# Autodesk Inventor assembly: Synchronous Belts Transmission
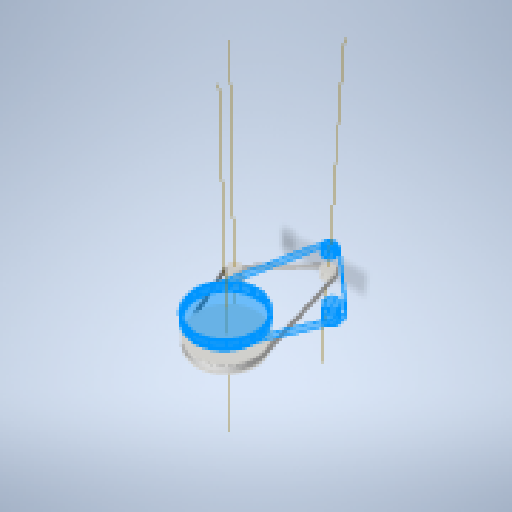
[picture p0: Inventor's stored thumbnail of the model, 512x512]
Saved by Autodesk Inventor 2024 (Build 280153000, 153)
## iProperties
ClientObjectVersion: 1
Created: 2024-01-05
Part Number: Synchronous Belts Transmission
Document SubType Name: Assembly
Designer: MaartenGeorgesBuelen
Author: MaartenGeorgesBuelen
## Documents named in this file (5)
- C:\Users\MaartenGeorgesBuelen\Documents\Inventor\robot arm\base\Design Accelerator\Synchronous Belts Transmission3.iam
- C:\Users\MaartenGeorgesBuelen\Documents\Inventor\robot arm\base\Design Accelerator\Synchronous Belt3.ipt
- C:\Users\MaartenGeorgesBuelen\Documents\Inventor\robot arm\base\Design Accelerator\Synchronous Pulley13.ipt
- C:\Users\MaartenGeorgesBuelen\Documents\Inventor\robot arm\base\Design Accelerator\Synchronous Pulley23.ipt
- C:\Users\MaartenGeorgesBuelen\Documents\Inventor\robot arm\base\Design Accelerator\Synchronous Pulley32.ipt
## Components (4 placed, 4 different names)
1. Synchronous Belt:1 — Flush:1, Mate:1, Mate:2, Flush:2, Mate:3, Mate:4, Flush:3, Mate:5, Mate:6
2. Synchronous Pulley1:1 — Flush:1, Mate:1, Mate:2, Rotation:1, Rotation:2
3. Synchronous Pulley2:1 — Flush:2, Mate:3, Rotation:1, Mate:4
4. Synchronous Pulley3:1 — Flush:3, Mate:5, Rotation:2, Mate:6
## Relationships (11: Mate 6, Flush 3, RelateRotation 2)
- Flush:1: Synchronous Belt:1 ↔ Synchronous Pulley1:1
- Mate:1: Synchronous Belt:1 ↔ Synchronous Pulley1:1
- Mate:2: Synchronous Belt:1 ↔ Synchronous Pulley1:1
- Flush:2: Synchronous Belt:1 ↔ Synchronous Pulley2:1
- Mate:3: Synchronous Belt:1 ↔ Synchronous Pulley2:1
- Rotation:1 [RelateRotation] (4 ul): Synchronous Pulley1:1 ↔ Synchronous Pulley2:1
- Mate:4: Synchronous Belt:1 ↔ Synchronous Pulley2:1
- Flush:3: Synchronous Belt:1 ↔ Synchronous Pulley3:1
- Mate:5: Synchronous Belt:1 ↔ Synchronous Pulley3:1
- Rotation:2 [RelateRotation] (1.25 ul): Synchronous Pulley1:1 ↔ Synchronous Pulley3:1
- Mate:6: Synchronous Belt:1 ↔ Synchronous Pulley3:1
